# Autodesk Inventor assembly: MIRleft脚右
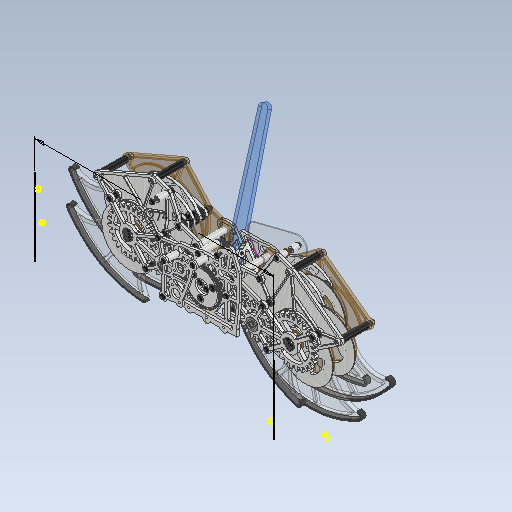
[picture p0: Inventor's stored thumbnail of the model, 512x512]
Saved by Autodesk Inventor 2020.2 (Build 242310000, 310)
## iProperties
Created: 2020-04-15
Part Number: MIRleft脚右
Document SubType Name: Assembly
Designer: aoyama
Mass: 561.522 g
Surface Area: 3837.69 cm^2
Volume: 258.191 cm^3
Density: 2.17483 g/cm^3
Author: aoyama
## Documents named in this file (17)
- C:\Users\aoyam\Desktop\SRDC_local\Inventor\二年機\Geminiβ\脚\MIR達\MIRleft脚右.iam
- C:\Users\aoyam\Desktop\SRDC_local\Inventor\二年機\Geminiβ\脚\MIR達\MIRleft脚四半.iam
- C:\Users\aoyam\Desktop\SRDC_local\Inventor\二年機\Geminiβ\脚\中間ユニット\MIR達\MIRleft中間ユニット.iam
- C:\Users\aoyam\Desktop\SRDC_local\Inventor\二年機\Geminiβ\汎用部品\MIR達\MIRleftオイレスFd6D8L3.ipt
- C:\Users\aoyam\Desktop\SRDC_local\Inventor\二年機\Geminiβ\脚\MIR達\MIRleftMIRright脚四半.iam
- C:\Users\aoyam\Desktop\SRDC_local\Inventor\二年機\Geminiβ\汎用部品\MIR達\MIRleftワッシャD7d3m0.5.ipt
- C:\Users\aoyam\Desktop\SRDC_local\Inventor\二年機\Geminiβ\汎用部品\MIR達\MIRleftスペーサーM3L8アルミ.ipt
- C:\Users\aoyam\Desktop\SRDC_local\Inventor\二年機\Geminiβ\汎用部品\MIR達\MIRleftスペーサー中空M3L8アルミ.ipt
- C:\Users\aoyam\Desktop\SRDC_local\Inventor\二年機\Geminiβ\汎用部品\MIR達\MIRleftネジボタンM3L6.ipt
- C:\Users\aoyam\Desktop\SRDC_local\Inventor\二年機\Geminiβ\脚\MIR達\MIRleftダンパーガード.ipt
- C:\Users\aoyam\Desktop\SRDC_local\Inventor\二年機\Geminiβ\汎用部品\MIR達\MIRleftスペーサー中空M3L12アルミ.ipt
- C:\Users\aoyam\Desktop\SRDC_local\Inventor\二年機\Geminiβ\汎用部品\MIR達\MIRleftネジボタンM3L22.ipt
- C:\Users\aoyam\Desktop\SRDC_local\Inventor\二年機\Geminiβ\汎用部品\MIR達\MIRleftナットナイロンM3.ipt
- C:\Users\aoyam\Desktop\SRDC_local\Inventor\二年機\Geminiβ\汎用部品\MIR達\MIRleftネジボタンM3L8.ipt
- C:\Users\aoyam\Desktop\SRDC_local\Inventor\二年機\Geminiβ\汎用部品\ネジボタンM3L20.ipt
- C:\Users\aoyam\Desktop\SRDC_local\Inventor\二年機\Geminiβ\翼\WingUnit2L.iam
- C:\Users\aoyam\Desktop\SRDC_local\Inventor\二年機\Geminiβ\汎用部品\ネジ皿M3L4.ipt
## Components (18 placed, 16 different names)
1. MIRleft脚四半:1 [sub-assembly] — 挿入:37, 挿入:38, 挿入:56
2. MIRleft中間ユニット:1 [sub-assembly] — 挿入:13, 挿入:51, 挿入:52, 挿入:53, 挿入:54, 挿入:55, 挿入:56, 挿入:57, 挿入:58, 挿入:59
3. MIRleftオイレスFd6D8L3:1 — 挿入:51
4. MIRleftオイレスFd6D8L3:2 — 挿入:52
5. MIRleftMIRright脚四半:1 [sub-assembly] — メイト:1, 挿入:39, 挿入:40, 挿入:57
6. MIRleftワッシャD7d3m0.5:1 — 挿入:5, 挿入:6
7. MIRleftスペーサーM3L8アルミ:1 — 挿入:5, 挿入:39
8. MIRleftスペーサー中空M3L8アルミ:1 — 挿入:6, 挿入:9
9. MIRleftネジボタンM3L6:1 — 挿入:40
10. MIRleftダンパーガード:1 — メイト:1, 挿入:9, 挿入:46
11. MIRleftスペーサー中空M3L12アルミ:1 — 挿入:12, 挿入:37
12. MIRleftネジボタンM3L22:1 — 挿入:12
13. MIRleftナットナイロンM3:1 — 挿入:38
14. MIRleftネジボタンM3L8:1 — 挿入:13
15. ネジボタンM3L20:1 — 挿入:46
16. WingUnit2L:1 [sub-assembly] — 挿入:53, 挿入:54, 挿入:55
17. ネジ皿M3L4:1 — 挿入:58
18. ネジ皿M3L4:2 — 挿入:59
## Relationships (20: Insert 19, Mate 1)
- 挿入:5 [Insert]: MIRleftワッシャD7d3m0.5:1 ↔ MIRleftスペーサーM3L8アルミ:1
- 挿入:6 [Insert] (5 mm): MIRleftワッシャD7d3m0.5:1 ↔ MIRleftスペーサー中空M3L8アルミ:1
- メイト:1 [Mate]: MIRleftMIRright脚四半:1 ↔ MIRleftダンパーガード:1
- 挿入:9 [Insert]: MIRleftスペーサー中空M3L8アルミ:1 ↔ MIRleftダンパーガード:1
- 挿入:12 [Insert] (5 mm): MIRleftスペーサー中空M3L12アルミ:1 ↔ MIRleftネジボタンM3L22:1
- 挿入:13 [Insert] (5 mm): MIRleft中間ユニット:1 ↔ MIRleftネジボタンM3L8:1
- 挿入:37 [Insert]: MIRleft脚四半:1 ↔ MIRleftスペーサー中空M3L12アルミ:1
- 挿入:38 [Insert]: MIRleft脚四半:1 ↔ MIRleftナットナイロンM3:1
- 挿入:39 [Insert]: MIRleftMIRright脚四半:1 ↔ MIRleftスペーサーM3L8アルミ:1
- 挿入:40 [Insert]: MIRleftMIRright脚四半:1 ↔ MIRleftネジボタンM3L6:1
- 挿入:46 [Insert]: MIRleftダンパーガード:1 ↔ ネジボタンM3L20:1
- 挿入:51 [Insert]: MIRleft中間ユニット:1 ↔ MIRleftオイレスFd6D8L3:1
- 挿入:52 [Insert]: MIRleft中間ユニット:1 ↔ MIRleftオイレスFd6D8L3:2
- 挿入:53 [Insert]: MIRleft中間ユニット:1 ↔ WingUnit2L:1
- 挿入:54 [Insert]: MIRleft中間ユニット:1 ↔ WingUnit2L:1
- 挿入:55 [Insert]: MIRleft中間ユニット:1 ↔ WingUnit2L:1
- 挿入:56 [Insert]: MIRleft脚四半:1 ↔ MIRleft中間ユニット:1
- 挿入:57 [Insert]: MIRleft中間ユニット:1 ↔ MIRleftMIRright脚四半:1
- 挿入:58 [Insert]: MIRleft中間ユニット:1 ↔ ネジ皿M3L4:1
- 挿入:59 [Insert]: MIRleft中間ユニット:1 ↔ ネジ皿M3L4:2
